# Autodesk Inventor assembly: leg_Left_ass
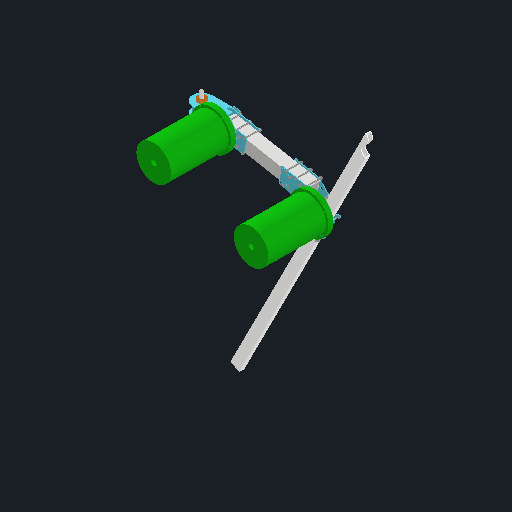
[picture p0: Inventor's stored thumbnail of the model, 512x512]
Saved by Autodesk Inventor 2026 (Build 300175000, 175)
## iProperties
Created: 2026-04-24
Part Number: leg_Left_ass
Document SubType Name: Assembly
Designer: user
Mass: 11319.9 g
Surface Area: 10601.7 cm^2
Volume: 6556.3 cm^3
Author: user
## Documents named in this file (6)
- C:\Users\user\vs_code_projects\ogonek-spider\physical-structure\cad\leg_Left_ass.iam
- C:\Users\user\vs_code_projects\ogonek-spider\physical-structure\cad\leg_tibea\leg_Left_tibea_ass.iam
- leg_Right_tibea_ass.iam
- C:\Users\user\vs_code_projects\ogonek-spider\physical-structure\cad\leg_femur\leg_Left_femur_ass.iam
- C:\Users\user\vs_code_projects\ogonek-spider\physical-structure\cad\leg_coxa\leg_Left_coxa_ass.iam
- C:\Users\user\vs_code_projects\ogonek-spider\physical-structure\cad\parametres.xlsx
## Components (3 placed, 3 different names)
1. leg_Left_tibea_ass:1 [sub-assembly] — С поворотом:1
2. leg_Left_femur_ass:1 [sub-assembly] — С поворотом:1, С поворотом:2
3. leg_Left_coxa_ass:1 [sub-assembly] — С поворотом:2, Совмещение:3
## Relationships (3: RevoluteJoint 2, Mate 1)
- С поворотом:1 [RevoluteJoint] (-10 mm): leg_Left_tibea_ass:1 ↔ leg_Left_femur_ass:1
- С поворотом:2 [RevoluteJoint] (-10 mm): leg_Left_femur_ass:1 ↔ leg_Left_coxa_ass:1
- Совмещение:3 [Mate]: leg_Left_coxa_ass:1
## Named parameters: tolerance_plazma = 0.1 mm, thickness_steel = 3 mm, d_main_screw_holes = 6.1 mm, d_main_shaft = 15 mm, thickness_profile_tibea = 3 mm, width_profile_tibea = 20 mm, hight_profile_tibea = 40 mm, length_profile_tibia = 800 mm, length_thorn_tibia = 400 mm, width_profile_femur = 50 mm, hight_profile_femur = 50 mm, thickness_profile_femur = 3 mm, length_profile_femur = 350 mm, width_shaft_shift = 35 mm, hight_shaft_shift = 37 mm, width_flattened_surface = 12 mm, length_coxa = 100 mm, hight_coxa = 40 mm, width_coxa = 80 mm, width_body_l3 = 120 mm, offset_body_l23 = 200 mm, width_body_l1 = 100 mm, offset_body_l12 = 60 mm, width_body_l2 = 150 mm, hight_ground_clearance = 500 mm
